# Autodesk Inventor assembly: s-assy-sun_gear
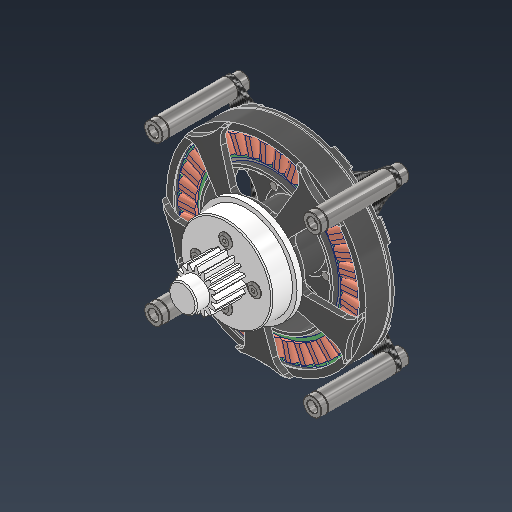
[picture p0: Inventor's stored thumbnail of the model, 512x512]
Saved by Autodesk Inventor 2021 (Build 250183000, 183)
## iProperties
Created: 2021-07-12
Part Number: s-assy-sun_gear
Document SubType Name: Assembly
Designer: yuta0
Mass: 337.358 g
Surface Area: 828.401 cm^2
Volume: 95.8223 cm^3
Density: 3.52066 g/cm^3
Author: yuta0
## Documents named in this file (10)
- C:\Users\yuta0\Desktop\catchrobo_robot\s-assy-sun_gear.iam
- C:\Users\yuta0\Desktop\catchrobo_robot\base16.ipt
- C:\Users\yuta0\Desktop\catchrobo_robot\ex8108.iam
- C:\Users\yuta0\Desktop\catchrobo_robot\CBSTNR3-12.ipt
- C:\Users\yuta0\Desktop\catchrobo_robot\s-assy-unit-magnet.iam
- C:\Users\yuta0\Desktop\catchrobo_robot\carbon_plate10.ipt
- C:\Users\yuta0\Desktop\catchrobo_robot\s-assy-unit-encoder.iam
- C:\Users\yuta0\Desktop\catchrobo_robot\unir-spacer2.ipt
- C:\Users\yuta0\Desktop\catchrobo_robot\unir-spacer6.ipt
- C:\Users\yuta0\Desktop\catchrobo_robot\CB4-6.ipt
## Components (25 placed, 9 different names)
1. s-assy-sun_gear:1 — メイト:13, メイト:14, メイト:15, メイト:16, メイト:17
2. s-assy-unit-magnet:1 [sub-assembly] — メイト:6
3. s-assy-unit-encoder:1 [sub-assembly] — メイト:20, メイト:32
4. ex8108:2 [sub-assembly] — メイト:12, メイト:13, メイト:14, メイト:15, メイト:18, メイト:21
5. unit-j2-plate2:1 — メイト:18, メイト:19, メイト:20, メイト:21, メイト:22, メイト:23, メイト:24, メイト:25, メイト:26, メイト:27
6. CBSTNR3-12:1 — メイト:16, メイト:17
7. unir-spacer2:1 — メイト:22, メイト:23, メイト:30, メイト:31
8. unir-spacer6:1 — メイト:30, メイト:31
9. CB4-6:1 — メイト:24, メイト:25
10. CB4-6:2 — メイト:26, メイト:27, メイト:32
11. CBSTNR3-12:2
12. unir-spacer2:2
13. unir-spacer6:2
14. CB4-6:3
15. CB4-6:4
16. CBSTNR3-12:3
17. unir-spacer2:3
18. unir-spacer6:3
19. CB4-6:5
20. CB4-6:6
21. CBSTNR3-12:4
22. unir-spacer2:4
23. unir-spacer6:4
24. CB4-6:7
25. CB4-6:8
## Component patterns: (4 elements, first: CBSTNR3-12:1 + unir-spacer2:1 + unir-spacer6:1 + CB4-6:1 + CB4-6:2)
## Relationships (21: Mate 21)
- メイト:6 [Mate]: s-assy-unit-magnet:1
- [Mate]: s-assy-unit-encoder:1 ↔ unit-j2-plate2:1
- メイト:12 [Mate]: ex8108:2
- メイト:13 [Mate]: s-assy-sun_gear:1 ↔ ex8108:2
- メイト:14 [Mate]: s-assy-sun_gear:1 ↔ ex8108:2
- メイト:15 [Mate]: s-assy-sun_gear:1 ↔ ex8108:2
- メイト:16 [Mate]: s-assy-sun_gear:1 ↔ CBSTNR3-12:1
- メイト:17 [Mate]: s-assy-sun_gear:1 ↔ CBSTNR3-12:1
- メイト:18 [Mate]: ex8108:2 ↔ unit-j2-plate2:1
- メイト:19 [Mate]: unit-j2-plate2:1
- メイト:20 [Mate]: s-assy-unit-encoder:1 ↔ unit-j2-plate2:1
- メイト:21 [Mate]: ex8108:2 ↔ unit-j2-plate2:1
- メイト:22 [Mate]: unit-j2-plate2:1 ↔ unir-spacer2:1
- メイト:23 [Mate]: unit-j2-plate2:1 ↔ unir-spacer2:1
- メイト:24 [Mate]: unit-j2-plate2:1 ↔ CB4-6:1
- メイト:25 [Mate]: unit-j2-plate2:1 ↔ CB4-6:1
- メイト:26 [Mate]: unit-j2-plate2:1 ↔ CB4-6:2
- メイト:27 [Mate]: unit-j2-plate2:1 ↔ CB4-6:2
- メイト:30 [Mate]: unir-spacer2:1 ↔ unir-spacer6:1
- メイト:31 [Mate]: unir-spacer2:1 ↔ unir-spacer6:1
- メイト:32 [Mate]: s-assy-unit-encoder:1 ↔ CB4-6:2
